# Autodesk Inventor assembly: chassis
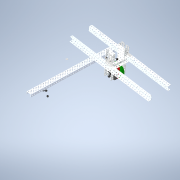
[picture p0: Inventor's stored thumbnail of the model, 180x180]
Saved by Autodesk Inventor 2021 (Build 250183000, 183)
## iProperties
Created: 2020-05-02
Part Number: chassis
Document SubType Name: Assembly
Designer: ajcar
Author: ajcar
## Documents named in this file (7)
- C:\Users\ajcar\Documents\vex_cad\chassis\chassis.iam
- C:\Users\ajcar\Documents\vex_cad\lib\Team 7479 Solidworks Library\Structure\C-Channel\C-Channel 1x2x1x35.ipt
- C:\Users\ajcar\Documents\vex_cad\tracking_wheels\tracking_wheels_v1.iam
- C:\Users\ajcar\Documents\vex_cad\lib\Team 7479 Solidworks Library\Structure\Misc\Angle Gusset.ipt
- C:\Users\ajcar\Documents\vex_cad\lib\Team 7479 Solidworks Library\Hardware\Stand-Offs & Couplers\Stand-Off .5in.ipt
- C:\Users\ajcar\Documents\vex_cad\lib\Team 7479 Solidworks Library\Hardware\Washers & Spacers\Plastic Spacer Thin.ipt
- C:\Users\ajcar\Documents\vex_cad\lib\Team 7479 Solidworks Library\Hardware\Washers & Spacers\Steel Washer.ipt
## Components (21 placed, 6 different names)
1. C-Channel 1x2x1x35:1 — Insert:6
2. C-Channel 1x2x1x35:2 — Angle:2, Mate:1, Angle:3, Mate:2, Angle:4, Insert:5, Insert:6, Insert:21
3. C-Channel 1x2x1x35:3 — Insert:4
4. tracking_wheels_v1:1 [sub-assembly] — Angle:2, Insert:14, Insert:15, Insert:18, Insert:19
5. Angle Gusset:1 — Mate:2, Angle:4, Insert:5, Tangent:1, Mate:5
6. Angle Gusset:2 — Mate:1, Angle:3, Insert:4
7. Stand-Off .5in:1 — Insert:9, Insert:18
8. Stand-Off .5in:2 — Insert:10, Insert:14
9. Plastic Spacer Thin:1
10. Plastic Spacer Thin:2 — Insert:10, Insert:11
11. Plastic Spacer Thin:3
12. Plastic Spacer Thin:4 — Insert:9, Tangent:2
13. Plastic Spacer Thin:5
14. Steel Washer:1 — Insert:11
15. Steel Washer:2
16. Stand-Off .5in:3 — Insert:15, Insert:16
17. Plastic Spacer Thin:6 — Insert:16, Insert:17
18. Steel Washer:3 — Insert:17
19. Stand-Off .5in:4 — Insert:19, Insert:20
20. Plastic Spacer Thin:7 — Insert:20, Tangent:1, Mate:5
21. Angle Gusset:5 — Insert:21, Tangent:2
## Relationships (25: Insert 16, Angle 4, Mate 3, Tangent 2)
- [Angle] (90 deg): C-Channel 1x2x1x35:1 ↔ C-Channel 1x2x1x35:2
- [Insert]: C-Channel 1x2x1x35:1 ↔ C-Channel 1x2x1x35:3
- [Insert]: C-Channel 1x2x1x35:1 ↔ C-Channel 1x2x1x35:3
- Angle:2 (0 deg): C-Channel 1x2x1x35:2 ↔ tracking_wheels_v1:1
- Mate:1: C-Channel 1x2x1x35:2 ↔ Angle Gusset:2
- Angle:3 (0 deg): C-Channel 1x2x1x35:2 ↔ Angle Gusset:2
- Insert:4: C-Channel 1x2x1x35:3 ↔ Angle Gusset:2
- Mate:2: C-Channel 1x2x1x35:2 ↔ Angle Gusset:1
- Angle:4 (0 deg): C-Channel 1x2x1x35:2 ↔ Angle Gusset:1
- Insert:5: C-Channel 1x2x1x35:2 ↔ Angle Gusset:1
- Insert:6: C-Channel 1x2x1x35:1 ↔ C-Channel 1x2x1x35:2
- Insert:9: Stand-Off .5in:1 ↔ Plastic Spacer Thin:4
- Insert:10: Stand-Off .5in:2 ↔ Plastic Spacer Thin:2
- Insert:11: Plastic Spacer Thin:2 ↔ Steel Washer:1
- Insert:14: tracking_wheels_v1:1 ↔ Stand-Off .5in:2
- Insert:15: tracking_wheels_v1:1 ↔ Stand-Off .5in:3
- Insert:16: Stand-Off .5in:3 ↔ Plastic Spacer Thin:6
- Insert:17: Plastic Spacer Thin:6 ↔ Steel Washer:3
- Insert:18: tracking_wheels_v1:1 ↔ Stand-Off .5in:1
- Insert:19: tracking_wheels_v1:1 ↔ Stand-Off .5in:4
- Insert:20: Stand-Off .5in:4 ↔ Plastic Spacer Thin:7
- Tangent:1: Angle Gusset:1 ↔ Plastic Spacer Thin:7
- Insert:21: C-Channel 1x2x1x35:2 ↔ Angle Gusset:5
- Tangent:2: Plastic Spacer Thin:4 ↔ Angle Gusset:5
- Mate:5: Angle Gusset:1 ↔ Plastic Spacer Thin:7
## Named parameters: d0_d1 = 90 deg, d1_d3 = 0 mm
